# Autodesk Inventor assembly: ProjectX
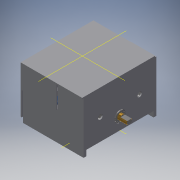
[picture p0: Inventor's stored thumbnail of the model, 180x180]
Saved by Autodesk Inventor 2019.4 (Build 234330000, 330)
## iProperties
Created: 2021-04-19
Part Number: ProjectX
Document SubType Name: Assembly
Designer: ville
Author: ville
## Documents named in this file (5)
- C:\Users\ville\OneDrive\Tiedostot\Inventor\Random\ProjectX.iam
- C:\Users\ville\OneDrive\Tiedostot\Inventor\Random\ProjectXBase.ipt
- C:\Users\ville\OneDrive\Tiedostot\Inventor\Random\ProjectXMotor.ipt
- C:\Users\ville\OneDrive\Tiedostot\Inventor\Random\arduino-nano-12.snapshot.1\Arduino Nano.ipt
- C:\Users\ville\OneDrive\Tiedostot\Inventor\Random\ProjectXBaseTop.ipt
## Components (4 placed, 4 different names)
1. ProjectXBase:1 — Mate:1, Mate:2, Mate:3, Mate:4, Mate:5, Flush:1, Mate:6, Flush:2
2. ProjectXMotor:1 — Mate:1, Mate:2, Mate:3
3. Arduino Nano:1 — Mate:4, Mate:5, Flush:2
4. ProjectXBaseTop:1 — Flush:1, Mate:6
## Relationships (8: Mate 6, Flush 2)
- Mate:1: ProjectXBase:1 ↔ ProjectXMotor:1
- Mate:2: ProjectXBase:1 ↔ ProjectXMotor:1
- Mate:3: ProjectXBase:1 ↔ ProjectXMotor:1
- Mate:4: ProjectXBase:1 ↔ Arduino Nano:1
- Mate:5: ProjectXBase:1 ↔ Arduino Nano:1
- Flush:1: ProjectXBase:1 ↔ ProjectXBaseTop:1
- Mate:6: ProjectXBase:1 ↔ ProjectXBaseTop:1
- Flush:2: ProjectXBase:1 ↔ Arduino Nano:1
